# Autodesk Inventor assembly: Base2
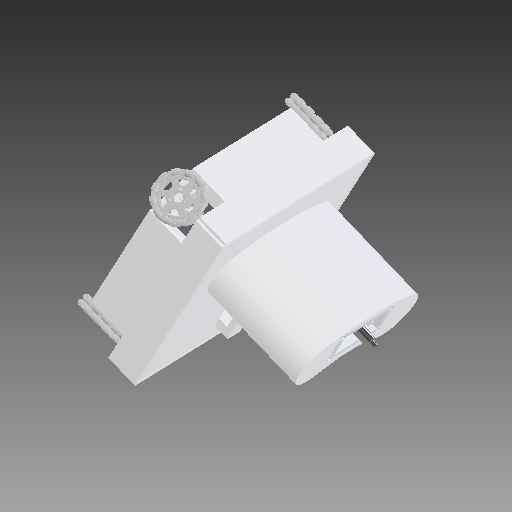
[picture p0: Inventor's stored thumbnail of the model, 512x512]
Saved by Autodesk Inventor 2017 SP1 (Build 210196100, 196)
## iProperties
Created: 2017-06-13
Part Number: Base2
Document SubType Name: Assembly
Designer: zallen
Author: zallen
## Documents named in this file (8)
- C:\Users\Zach\Documents\GitHub\cr-laundry-robot\src\Base 2\Base2.iam
- C:\Users\Zach\Documents\GitHub\cr-laundry-robot\src\Base 2\Chassis\Chassis.iam
- C:\Users\Zach\Documents\GitHub\cr-laundry-robot\lib\DC Motor with Encoder\Motor.ipt
- C:\Users\Zach\Documents\GitHub\cr-laundry-robot\lib\Omni Wheel 6in\217-2585.ipt
- C:\Users\Zach\Documents\GitHub\cr-laundry-robot\lib\Linear Actuator 450mm\LinearActuator450mm.iam
- C:\Users\Zach\Documents\GitHub\cr-laundry-robot\src\Base 2\Riser Base.ipt
- C:\Users\Zach\Documents\GitHub\cr-laundry-robot\src\Base 2\Top Cover.ipt
- C:\Users\Zach\Documents\GitHub\cr-laundry-robot\src\Base 2\Front Cover.ipt
## Components (16 placed, 7 different names)
1. Chassis:1 [sub-assembly] — Mate:1, Mate:2, Mate:3, Mate:4, Mate:5, Mate:6, Mate:7, Mate:8, Mate:10, Mate:12, Mate:14, Mate:16, Mate:17, Mate:18, Mate:19, Mate:20, Mate:23, Mate:25, Mate:28, Mate:29, Mate:30, Mate:33
2. Motor:1 — Mate:1, Mate:2, Mate:13
3. Motor:2 — Mate:7, Mate:8, Mate:9
4. Motor:3 — Mate:5, Mate:6, Mate:15
5. Motor:4 — Mate:3, Mate:4, Mate:11
6. 217-2585:1 — Mate:9, Mate:10
7. 217-2585:2 — Mate:11, Mate:12
8. 217-2585:3 — Mate:13, Mate:14
9. 217-2585:4 — Mate:15, Mate:16
10. LinearActuator450mm:1 [sub-assembly] — Mate:17
11. Riser Base:1 — Mate:18, Mate:19, Mate:20, Mate:21, Mate:22
12. Top Cover:1 — Mate:21, Mate:22, Mate:23, Mate:24, Mate:26, Mate:27, Mate:31, Mate:32, Mate:34
13. Front Cover:1 — Mate:24, Mate:25, Mate:26, Mate:35
14. Front Cover:2 — Mate:27, Mate:28, Mate:29
15. Front Cover:3 — Mate:33, Mate:34, Mate:35
16. Front Cover:4 — Mate:30, Mate:31, Mate:32
## Relationships (35: Mate 35)
- Mate:1: Chassis:1 ↔ Motor:1
- Mate:2: Chassis:1 ↔ Motor:1
- Mate:3: Chassis:1 ↔ Motor:4
- Mate:4: Chassis:1 ↔ Motor:4
- Mate:5: Chassis:1 ↔ Motor:3
- Mate:6: Chassis:1 ↔ Motor:3
- Mate:7: Chassis:1 ↔ Motor:2
- Mate:8: Chassis:1 ↔ Motor:2
- Mate:9: Motor:2 ↔ 217-2585:1
- Mate:10: Chassis:1 ↔ 217-2585:1
- Mate:11: Motor:4 ↔ 217-2585:2
- Mate:12: Chassis:1 ↔ 217-2585:2
- Mate:13: Motor:1 ↔ 217-2585:3
- Mate:14: Chassis:1 ↔ 217-2585:3
- Mate:15: Motor:3 ↔ 217-2585:4
- Mate:16: Chassis:1 ↔ 217-2585:4
- Mate:17: Chassis:1 ↔ LinearActuator450mm:1
- Mate:18: Chassis:1 ↔ Riser Base:1
- Mate:19: Chassis:1 ↔ Riser Base:1
- Mate:20: Chassis:1 ↔ Riser Base:1
- Mate:21: Riser Base:1 ↔ Top Cover:1
- Mate:22: Riser Base:1 ↔ Top Cover:1
- Mate:23: Chassis:1 ↔ Top Cover:1
- Mate:24: Top Cover:1 ↔ Front Cover:1
- Mate:25: Chassis:1 ↔ Front Cover:1
- Mate:26: Top Cover:1 ↔ Front Cover:1
- Mate:27: Top Cover:1 ↔ Front Cover:2
- Mate:28: Chassis:1 ↔ Front Cover:2
- Mate:29: Chassis:1 ↔ Front Cover:2
- Mate:30: Chassis:1 ↔ Front Cover:4
- Mate:31: Top Cover:1 ↔ Front Cover:4
- Mate:32: Top Cover:1 ↔ Front Cover:4
- Mate:33: Chassis:1 ↔ Front Cover:3
- Mate:34: Top Cover:1 ↔ Front Cover:3
- Mate:35: Front Cover:1 ↔ Front Cover:3
